# Autodesk Inventor assembly: FloatingIntake2
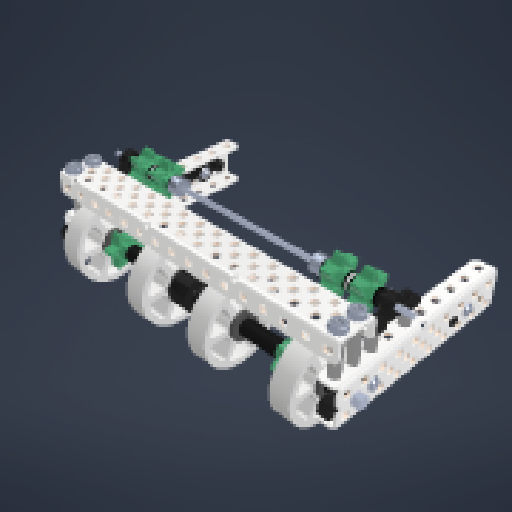
[picture p0: Inventor's stored thumbnail of the model, 512x512]
Saved by Autodesk Inventor 2023 (Build 270158000, 158)
## iProperties
Created: 2022-10-30
Part Number: FloatingIntake2
Document SubType Name: Assembly
Designer: alex
Author: alex
## Documents named in this file (32)
- C:\Users\alex\Documents\GitHub\4067X_spin_up_cad\FloatingIntake2.iam
- C:\Users\alex\Documents\GitHub\4067X_spin_up_cad\WithAdapter2Inch.iam
- C:\Users\alex\Documents\GitHub\4067X_spin_up_cad\Library\Structure\C-Channels\Aluminum 1x2x1\Alu C 1x2x1x10.ipt
- C:\Users\alex\Documents\GitHub\4067X_spin_up_cad\Library\Structure\Standoff\Standoff 1.00.ipt
- C:\Users\alex\Documents\GitHub\4067X_spin_up_cad\Library\Structure\Standoff.ipt
- C:\Users\alex\Documents\GitHub\4067X_spin_up_cad\Library\Structure\C-Channels\Aluminum 1x2x1\Alu C 1x2x1x16.ipt
- C:\Users\alex\Documents\GitHub\4067X_spin_up_cad\Library\Motion\Sprockets\HS 6T Sprocket, No Insert.ipt
- C:\Users\alex\Documents\GitHub\4067X_spin_up_cad\Library\Motion\Shaft HS\Shaft HS\Shaft HS 8.5 in.ipt
- C:\Users\alex\Documents\GitHub\4067X_spin_up_cad\Library\Motion\Shaft HS\Shaft HS.ipt
- C:\Users\alex\Documents\GitHub\4067X_spin_up_cad\Library\Motion\Shaft HS\HS Bearing Flat.ipt
- C:\Users\alex\Documents\GitHub\4067X_spin_up_cad\Library\Structure\Hardware\Screw Steel - Star\SScrew Star Smooth .500.ipt
- C:\Users\alex\Documents\GitHub\4067X_spin_up_cad\Library\Structure\Hardware\Screw Steel - Star.ipt
- C:\Users\alex\Documents\GitHub\4067X_spin_up_cad\Library\Structure\Hardware\Nut Thin Nylock.ipt
- C:\Users\alex\Documents\GitHub\4067X_spin_up_cad\Library\Motion\1-Post Bearing Flat Hex Retainer.ipt
- C:\Users\alex\Documents\GitHub\4067X_spin_up_cad\Library\Structure\Hardware\Nut Nylock.ipt
- C:\Users\alex\Documents\GitHub\4067X_spin_up_cad\Library\Structure\Hardware\Screw Steel - Star\SScrew Star Smooth .375.ipt
- C:\Users\alex\Documents\GitHub\4067X_spin_up_cad\Library\Motion\Shaft HS\HS Spacer\HSpacer .1250.ipt
- C:\Users\alex\Documents\GitHub\4067X_spin_up_cad\Library\Motion\Shaft HS\HS Spacer.ipt
- C:\Users\alex\Documents\GitHub\4067X_spin_up_cad\Library\Structure\Hardware\Screw Steel - Star\SScrew Star Smooth 1.250.ipt
- C:\Users\alex\Documents\GitHub\4067X_spin_up_cad\Library\Structure\Hardware\Nut Keps.ipt
- C:\Users\alex\Documents\GitHub\4067X_spin_up_cad\Library\Structure\Standoff\Standoff .50.ipt
- C:\Users\alex\Documents\GitHub\4067X_spin_up_cad\Library\Motion\Pillow Bearing Block.ipt
- C:\Users\alex\Documents\GitHub\4067X_spin_up_cad\Library\Motion\Shaft LS\Shaft LS 8.5 in.ipt
- C:\Users\alex\Documents\GitHub\4067X_spin_up_cad\Library\Motion\Shaft LS.ipt
- C:\Users\alex\Documents\GitHub\4067X_spin_up_cad\Library\Motion\Sprockets\HS 6T Sprocket, Square.ipt
- C:\Users\alex\Documents\GitHub\4067X_spin_up_cad\Library\Motion\Spacers\Spacer Nylon .375 OD\NSpacer .375 OD x .125.ipt
- C:\Users\alex\Documents\GitHub\4067X_spin_up_cad\Library\Motion\Spacers\Spacer Nylon .375 OD.ipt
- C:\Users\alex\Documents\GitHub\4067X_spin_up_cad\Library\Motion\Spacers\Washer Teflon\TWasher .375 OD x .06250.ipt
- C:\Users\alex\Documents\GitHub\4067X_spin_up_cad\Library\Motion\Spacers\Washer Teflon.ipt
- C:\Users\alex\Documents\GitHub\4067X_spin_up_cad\Library\Motion\Shaft Collar with Set Screw.ipt
- C:\Users\alex\Documents\GitHub\4067X_spin_up_cad\Library\Motion\Shaft HS\HS Spacer\HSpacer .5000.ipt
- C:\Users\alex\Documents\GitHub\4067X_spin_up_cad\Library\Motion\Shaft HS\HS Shaft Collar.ipt
## Components (59 placed, 24 different names)
1. WithAdapter2Inch:1 [sub-assembly] — Insert:34, Insert:35
2. Alu C 1x2x1x10:1 — Flush:1, Insert:23, Insert:24, Insert:38, Insert:39
3. Alu C 1x2x1x10:2 — Flush:1, Insert:21, Mate:6, Insert:22, Insert:25, Insert:26, Insert:42, Insert:43
4. Standoff 1.00:1
5. Standoff 1.00:2
6. Standoff 1.00:3
7. Standoff 1.00:4
8. Alu C 1x2x1x16:1 — Insert:27, Insert:28, Insert:29, Insert:30
9. Shaft HS 8.5 in:1
10. HS Bearing Flat:1 — Insert:17
11. SScrew Star Smooth .500:1
12. Nut Thin Nylock:1
13. 1-Post Bearing Flat Hex Retainer:1
14. Nut Nylock:1
15. SScrew Star Smooth .375:2
16. SScrew Star Smooth .375:3
17. Nut Nylock:2
18. 1-Post Bearing Flat Hex Retainer:2
19. HSpacer .1250:1 — Insert:17, Insert:34
20. HS Bearing Flat:2 — Insert:21, Mate:6, Insert:31
21. Nut Thin Nylock:2
22. SScrew Star Smooth .500:4 — Insert:22
23. SScrew Star Smooth 1.250:5 — Insert:23
24. SScrew Star Smooth 1.250:6 — Insert:24
25. SScrew Star Smooth 1.250:7 — Insert:25
26. SScrew Star Smooth 1.250:8 — Insert:26
27. Nut Keps:1 — Insert:27
28. Nut Keps:2 — Insert:28
29. Nut Keps:3 — Insert:29
30. Nut Keps:4 — Insert:30
31. HSpacer .1250:2 — Insert:31, Insert:36
32. WithAdapter2Inch:2 [sub-assembly] — Insert:36, Insert:37
33. HS 6T Sprocket, No Insert:3 — Insert:35, Insert:71
34. HS 6T Sprocket, No Insert:4 — Insert:37, Insert:66
35. Standoff .50:5 — Insert:38, Insert:40
36. Standoff .50:6 — Insert:39, Mate:7
37. Pillow Bearing Block:1 — Insert:40, Mate:7, Insert:58, Flush:3
38. Standoff .50:7 — Insert:42
39. Standoff .50:8 — Insert:43
40. Pillow Bearing Block:2 — Insert:61
41. Shaft LS 8.5 in:1 — Mate:9, Mate:10, Flush:3
42. TWasher .375 OD x .06250:1 — Insert:60, Insert:64
43. HS 6T Sprocket, Square:3 — Insert:53, Insert:57
44. Shaft Collar with Set Screw:2 — Insert:53
45. TWasher .375 OD x .06250:3 — Insert:57, Insert:63
46. NSpacer .375 OD x .125:3 — Insert:58, Insert:59
47. HS 6T Sprocket, Square:5 — Insert:59, Insert:60
48. NSpacer .375 OD x .125:4 — Insert:61, Insert:62
49. HS 6T Sprocket, Square:6 — Insert:62, Insert:63
50. HS 6T Sprocket, Square:7 — Mate:9, Mate:10, Insert:64, Insert:65
51. Shaft Collar with Set Screw:3 — Insert:65
52. HSpacer .5000:3 — Insert:66, Insert:67
53. HSpacer .5000:4 — Insert:67, Insert:68
54. WithAdapter2Inch:3 [sub-assembly] — Insert:68
55. HSpacer .5000:5 — Insert:71
56. HSpacer .5000:6
57. WithAdapter2Inch:4 [sub-assembly]
58. HS Shaft Collar:1
59. HS Shaft Collar:2
## Relationships (71: Insert 55, Mate 12, Flush 3, Angle 1)
- [Mate]: WithAdapter2Inch:1 ↔ Alu C 1x2x1x10:1
- [Angle] (0 deg): Alu C 1x2x1x10:1 ↔ Alu C 1x2x1x10:2
- [Insert]: Alu C 1x2x1x10:1 ↔ Standoff 1.00:1
- [Insert]: Alu C 1x2x1x10:1 ↔ Standoff 1.00:2
- [Insert]: Alu C 1x2x1x10:2 ↔ Standoff 1.00:3
- [Insert]: Alu C 1x2x1x10:2 ↔ Standoff 1.00:4
- [Insert]: Standoff 1.00:3 ↔ Alu C 1x2x1x16:1
- [Insert]: Standoff 1.00:1 ↔ Alu C 1x2x1x16:1
- Flush:1: Alu C 1x2x1x10:1 ↔ Alu C 1x2x1x10:2
- [Mate]: Alu C 1x2x1x10:2 ↔ Shaft HS 8.5 in:1
- [Flush] (-5.08 mm): Alu C 1x2x1x10:1 ↔ Shaft HS 8.5 in:1
- [Insert]: Alu C 1x2x1x10:1 ↔ HS Bearing Flat:1
- [Mate]: Alu C 1x2x1x10:1 ↔ HS Bearing Flat:1
- [Insert]: Alu C 1x2x1x10:1 ↔ SScrew Star Smooth .500:1
- [Insert]: HS Bearing Flat:1 ↔ Nut Thin Nylock:1
- [Insert]: 1-Post Bearing Flat Hex Retainer:1 ↔ Nut Nylock:1
- [Insert]: Alu C 1x2x1x10:2 ↔ 1-Post Bearing Flat Hex Retainer:1
- [Mate]: Alu C 1x2x1x10:2 ↔ 1-Post Bearing Flat Hex Retainer:1
- [Insert]: Alu C 1x2x1x10:2 ↔ SScrew Star Smooth .375:2
- [Insert]: Alu C 1x2x1x10:1 ↔ 1-Post Bearing Flat Hex Retainer:2
- [Mate]: Alu C 1x2x1x10:1 ↔ 1-Post Bearing Flat Hex Retainer:2
- [Insert]: Alu C 1x2x1x10:1 ↔ SScrew Star Smooth .375:3
- [Insert]: Nut Nylock:2 ↔ 1-Post Bearing Flat Hex Retainer:2
- Insert:17: HS Bearing Flat:1 ↔ HSpacer .1250:1
- [Insert]: HS Bearing Flat:2 ↔ Nut Thin Nylock:2
- Insert:21: Alu C 1x2x1x10:2 ↔ HS Bearing Flat:2
- Mate:6: Alu C 1x2x1x10:2 ↔ HS Bearing Flat:2
- Insert:22: Alu C 1x2x1x10:2 ↔ SScrew Star Smooth .500:4
- Insert:23: Alu C 1x2x1x10:1 ↔ SScrew Star Smooth 1.250:5
- Insert:24: Alu C 1x2x1x10:1 ↔ SScrew Star Smooth 1.250:6
- Insert:25: Alu C 1x2x1x10:2 ↔ SScrew Star Smooth 1.250:7
- Insert:26: Alu C 1x2x1x10:2 ↔ SScrew Star Smooth 1.250:8
- Insert:27: Alu C 1x2x1x16:1 ↔ Nut Keps:1
- Insert:28: Alu C 1x2x1x16:1 ↔ Nut Keps:2
- Insert:29: Alu C 1x2x1x16:1 ↔ Nut Keps:3
- Insert:30: Alu C 1x2x1x16:1 ↔ Nut Keps:4
- Insert:31: HS Bearing Flat:2 ↔ HSpacer .1250:2
- Insert:34: WithAdapter2Inch:1 ↔ HSpacer .1250:1
- Insert:35: WithAdapter2Inch:1 ↔ HS 6T Sprocket, No Insert:3
- Insert:36: HSpacer .1250:2 ↔ WithAdapter2Inch:2
- Insert:37: WithAdapter2Inch:2 ↔ HS 6T Sprocket, No Insert:4
- Insert:38: Alu C 1x2x1x10:1 ↔ Standoff .50:5
- Insert:39: Alu C 1x2x1x10:1 ↔ Standoff .50:6
- Insert:40: Standoff .50:5 ↔ Pillow Bearing Block:1
- Mate:7: Standoff .50:6 ↔ Pillow Bearing Block:1
- [Insert]: Standoff .50:7 ↔ Pillow Bearing Block:2
- [Mate]: Standoff .50:8 ↔ Pillow Bearing Block:2
- Insert:42: Alu C 1x2x1x10:2 ↔ Standoff .50:7
- Insert:43: Alu C 1x2x1x10:2 ↔ Standoff .50:8
- Insert:53: HS 6T Sprocket, Square:3 ↔ Shaft Collar with Set Screw:2
- Insert:57: HS 6T Sprocket, Square:3 ↔ TWasher .375 OD x .06250:3
- Insert:58: Pillow Bearing Block:1 ↔ NSpacer .375 OD x .125:3
- Insert:59: NSpacer .375 OD x .125:3 ↔ HS 6T Sprocket, Square:5
- Insert:60: TWasher .375 OD x .06250:1 ↔ HS 6T Sprocket, Square:5
- Insert:61: Pillow Bearing Block:2 ↔ NSpacer .375 OD x .125:4
- Insert:62: NSpacer .375 OD x .125:4 ↔ HS 6T Sprocket, Square:6
- Insert:63: TWasher .375 OD x .06250:3 ↔ HS 6T Sprocket, Square:6
- Mate:9: Shaft LS 8.5 in:1 ↔ HS 6T Sprocket, Square:7
- Mate:10: Shaft LS 8.5 in:1 ↔ HS 6T Sprocket, Square:7
- Insert:64: TWasher .375 OD x .06250:1 ↔ HS 6T Sprocket, Square:7
- Flush:3 (-9.525 mm): Pillow Bearing Block:1 ↔ Shaft LS 8.5 in:1
- Insert:65: HS 6T Sprocket, Square:7 ↔ Shaft Collar with Set Screw:3
- Insert:66: HS 6T Sprocket, No Insert:4 ↔ HSpacer .5000:3
- Insert:67: HSpacer .5000:3 ↔ HSpacer .5000:4
- Insert:68: HSpacer .5000:4 ↔ WithAdapter2Inch:3
- [Insert]: HSpacer .5000:5 ↔ HSpacer .5000:6
- [Insert]: HSpacer .5000:6 ↔ WithAdapter2Inch:4
- Insert:71: HS 6T Sprocket, No Insert:3 ↔ HSpacer .5000:5
- [Mate]: Shaft HS 8.5 in:1 ↔ HS Shaft Collar:1
- [Mate]: WithAdapter2Inch:4 ↔ HS Shaft Collar:1
- [Insert]: WithAdapter2Inch:3 ↔ HS Shaft Collar:2
## Named parameters: d174_d168 = 0 mm, d27_d182 = 0 mm, d51_d49 = 0 mm, d52_d50 = 0 mm, d85_d83 = 0 mm, d86_d84 = 0 mm
